# Autodesk Inventor assembly: CL5-100
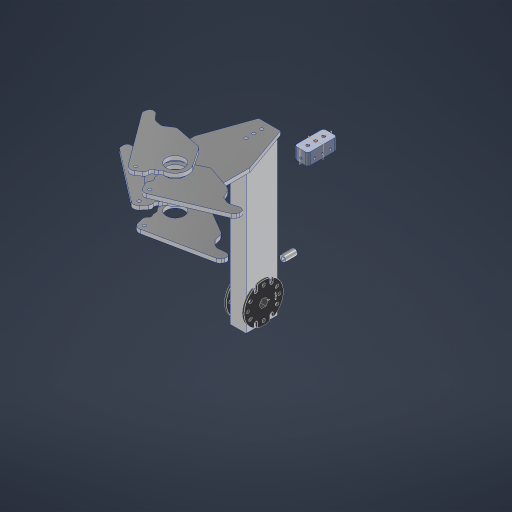
[picture p0: Inventor's stored thumbnail of the model, 512x512]
Saved by Autodesk Inventor 2023.4 (Build 274418000, 418)
## iProperties
Created: 2025-02-04
Part Number: CL5-100
Document SubType Name: Assembly
Designer: brand
Author: brand
## Documents named in this file (9)
- C:\Users\brand\OneDrive\Documents\GitHub\robotics 23\2025-ReefScape---CAD\Climber\CL5\CL5-100.iam
- C:\Users\brand\OneDrive\Documents\GitHub\robotics 23\2025-ReefScape---CAD\Field Items\Full Field\FE-2025\GE-25201.iam
- C:\Users\brand\OneDrive\Documents\GitHub\robotics 23\2025-ReefScape---CAD\Climber\CL4\02_Barb Assembly (1)\02_Barb Assembly (1).iam
- C:\Users\brand\OneDrive\Documents\GitHub\robotics 23\2025-ReefScape---CAD\COMMON PARTS\HUBS\WCP-1388.ipt
- C:\Users\brand\OneDrive\Documents\GitHub\robotics 23\2025-ReefScape---CAD\Climber\CL5\CL5-001.ipt
- C:\Users\brand\OneDrive\Documents\GitHub\robotics 23\2025-ReefScape---CAD\Elevator\EL2\EL2-005.ipt
- C:\Users\brand\OneDrive\Documents\GitHub\robotics 23\2025-ReefScape---CAD\Climber\CL5\CL5-002.ipt
- C:\Users\brand\OneDrive\Documents\GitHub\robotics 23\2025-ReefScape---CAD\Climber\CL5\CL5-003.ipt
- C:\Users\brand\OneDrive\Documents\GitHub\robotics 23\2025-ReefScape---CAD\Climber\CL5\CL5-004.ipt
## Components (12 placed, 8 different names)
1. CL5-001:1 — Mate:7, Flush:6, Flush:7, Insert:2, Mate:14, Insert:3, Mate:15, Mate:16, Mate:17, Flush:8, Flush:9
2. GE-25201:1 [sub-assembly] — Mate:7
3. 02_Barb Assembly (1):1 [sub-assembly] — Flush:6, Flush:7
4. WCP-1388:1 — Insert:2, Mate:14
5. WCP-1388:2 — Insert:3, Mate:15
6. EL2-005:1
7. CL5-002:1 — Mate:17, Flush:8, Mate:18, Mate:19, Mate:20, Mate:21, Flush:9
8. CL5-003:1 — Mate:18
9. CL5-004:1
10. CL5-003:2 — Mate:21
11. CL5-003:4 — Mate:19
12. CL5-003:5 — Mate:20
## Relationships (15: Mate 9, Flush 4, Insert 2)
- Mate:7: CL5-001:1 ↔ GE-25201:1
- Flush:6: CL5-001:1 ↔ 02_Barb Assembly (1):1
- Flush:7: CL5-001:1 ↔ 02_Barb Assembly (1):1
- Insert:2: CL5-001:1 ↔ WCP-1388:1
- Mate:14: CL5-001:1 ↔ WCP-1388:1
- Insert:3: CL5-001:1 ↔ WCP-1388:2
- Mate:15: CL5-001:1 ↔ WCP-1388:2
- Mate:16: CL5-001:1
- Mate:17: CL5-001:1 ↔ CL5-002:1
- Flush:8: CL5-001:1 ↔ CL5-002:1
- Mate:18: CL5-002:1 ↔ CL5-003:1
- Mate:19: CL5-002:1 ↔ CL5-003:4
- Mate:20: CL5-002:1 ↔ CL5-003:5
- Mate:21: CL5-002:1 ↔ CL5-003:2
- Flush:9: CL5-001:1 ↔ CL5-002:1
